# Autodesk Inventor assembly: Mao-robotica-alpha
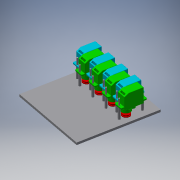
[picture p0: Inventor's stored thumbnail of the model, 180x180]
Saved by Autodesk Inventor 2018 (Build 220112000, 112)
## iProperties
Created: 2017-06-01
Part Number: Mao-robotica-alpha
Material: Genérico
Document SubType Name: Assembly
Designer: Vitor
Author: Vitor
## Documents named in this file (4)
- C:\Users\Vitor\Documents\Autodesk\Mao-Robotica\Mao-robotica-alpha.iam
- C:\Users\Vitor\Documents\Autodesk\Mao-Robotica\Palma.ipt
- C:\Users\Vitor\Documents\Autodesk\Mao-Robotica\Motor.ipt
- C:\Users\Vitor\Documents\Autodesk\Mao-Robotica\Polia.ipt
## Components (17 placed, 3 different names)
1. Palma:1 — Inserir:2, Inserir:3, Inserir:5, Inserir:6, Inserir:13, Inserir:14, Inserir:15, Inserir:16, Inserir:17, Inserir:18, Inserir:19, Inserir:20, Inserir:21, Inserir:22, Inserir:23, Inserir:24
2. Motor:1 — Inserir:7, Inserir:15, Inserir:16
3. Motor:2 — Inserir:1, Inserir:2, Inserir:3
4. Motor:3 — Inserir:8, Inserir:13, Inserir:14
5. Motor:4 — Inserir:9, Inserir:17, Inserir:18
6. Motor:5 — Inserir:10, Inserir:19, Inserir:20
7. Motor:6 — Inserir:11, Inserir:21, Inserir:22
8. Motor:7 — Inserir:12, Inserir:23, Inserir:24
9. Motor:8 — Inserir:4, Inserir:5, Inserir:6
10. Polia:1 — Inserir:4
11. Polia:2 — Inserir:12
12. Polia:3 — Inserir:11
13. Polia:4 — Inserir:10
14. Polia:5 — Inserir:9
15. Polia:6 — Inserir:8
16. Polia:7 — Inserir:7
17. Polia:8 — Inserir:1
## Relationships (24: Insert 24)
- Inserir:1: Motor:2 ↔ Polia:8
- Inserir:2: Palma:1 ↔ Motor:2
- Inserir:3: Palma:1 ↔ Motor:2
- Inserir:4: Motor:8 ↔ Polia:1
- Inserir:5: Palma:1 ↔ Motor:8
- Inserir:6: Palma:1 ↔ Motor:8
- Inserir:7: Motor:1 ↔ Polia:7
- Inserir:8: Motor:3 ↔ Polia:6
- Inserir:9: Motor:4 ↔ Polia:5
- Inserir:10: Motor:5 ↔ Polia:4
- Inserir:11: Motor:6 ↔ Polia:3
- Inserir:12: Motor:7 ↔ Polia:2
- Inserir:13: Palma:1 ↔ Motor:3
- Inserir:14: Palma:1 ↔ Motor:3
- Inserir:15: Palma:1 ↔ Motor:1
- Inserir:16: Palma:1 ↔ Motor:1
- Inserir:17: Palma:1 ↔ Motor:4
- Inserir:18: Palma:1 ↔ Motor:4
- Inserir:19: Palma:1 ↔ Motor:5
- Inserir:20: Palma:1 ↔ Motor:5
- Inserir:21: Palma:1 ↔ Motor:6
- Inserir:22: Palma:1 ↔ Motor:6
- Inserir:23: Palma:1 ↔ Motor:7
- Inserir:24: Palma:1 ↔ Motor:7
